# Autodesk Inventor assembly: Assembly_Cube_Z_Focus_MGN_NEMA_captive_v3
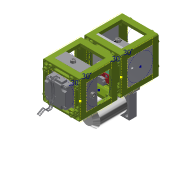
[picture p0: Inventor's stored thumbnail of the model, 180x180]
Saved by Autodesk Inventor 2022 (Build 260153000, 153)
## iProperties
Created: 2021-04-25
Part Number: Assembly_Cube_Z_Focus_MGN_NEMA_captive_v3
Document SubType Name: Assembly
Designer: diederichbenedict
Author: diederichbenedict
## Documents named in this file (17)
- C:\Users\diederichbenedict\Dropbox\Dokumente\Promotion\PROJECTS\UC2\02_CAD\INVENTOR\uc2_v3\Assembly_Cube_Z_Focus_MGN_NEMA_captive_v3.iam
- C:\Users\diederichbenedict\Dropbox\Dokumente\Promotion\PROJECTS\UC2\02_CAD\INVENTOR\uc2_v3\Assembly_Cube_empty_IM_v3.iam
- C:\Users\diederichbenedict\Dropbox\Dokumente\Promotion\PROJECTS\UC2\02_CAD\INVENTOR\uc2_v3\00_MGN12H, LINEAR GUIDE BLOCK.ipt
- C:\Users\diederichbenedict\Dropbox\Dokumente\Promotion\PROJECTS\UC2\02_CAD\INVENTOR\uc2_v3\00_NEMA11.ipt
- C:\Users\diederichbenedict\Dropbox\Dokumente\Promotion\PROJECTS\UC2\02_CAD\INVENTOR\uc2_v3\30_Cube_Z_Focus_MGN_NEMA_rail.ipt
- C:\Users\diederichbenedict\Dropbox\Dokumente\Promotion\PROJECTS\UC2\02_CAD\INVENTOR\uc2_v3\30_Cube_Z_Focus_MGN_NEMA_Motorsupport_centered.ipt
- C:\Users\diederichbenedict\Dropbox\Dokumente\Promotion\PROJECTS\UC2\02_CAD\INVENTOR\uc2_v3\30_Cube_Cube_Z_Focus_MGN_NEMA_belt_pushing_slide_v3.ipt
- C:\Users\diederichbenedict\Dropbox\Dokumente\Promotion\PROJECTS\UC2\02_CAD\INVENTOR\uc2_v3\30_Cube_Z_Focus_MGN_NEMA_base_belt_pushing_v3.ipt
- C:\Users\diederichbenedict\Dropbox\Dokumente\Promotion\PROJECTS\UC2\02_CAD\INVENTOR\uc2_v3\30_Cube_Z_Focus_MGN_NEMA_Motorcoupling_Captive_v3.ipt
- C:\Users\diederichbenedict\Documents\Inventor\Content Center Files\R2022\de-DE\DIN 912\DIN 912 - M3 x 0.5 x 30 x 18.ipt
- C:\Users\diederichbenedict\Documents\Inventor\Content Center Files\R2022\de-DE\DIN 912\DIN 912 - M3 x 0.5 x 16 x 14.75.ipt
- C:\Users\diederichbenedict\Documents\Inventor\Content Center Files\R2022\de-DE\DIN EN ISO 4032\DIN EN ISO 4032 - M3.ipt
- C:\Users\diederichbenedict\Documents\Inventor\Content Center Files\R2022\de-DE\DIN 912\DIN 912 - M3 x 0.5 x 8 x 6.75.ipt
- C:\Users\diederichbenedict\Dropbox\Dokumente\Promotion\PROJECTS\UC2\02_CAD\INVENTOR\uc2_v3\30_Cube_Z_Focus_MGN_NEMA_adapter_RMS.ipt
- C:\Users\diederichbenedict\Dropbox\Dokumente\Promotion\PROJECTS\UC2\02_CAD\INVENTOR\uc2_v3\00_Microscope_Objective_Lens10x.ipt
- C:\Users\diederichbenedict\Documents\Inventor\Content Center Files\R2022\de-DE\DIN 913\DIN 913 - M3 x 8.ipt
- C:\Users\diederichbenedict\Dropbox\Dokumente\Promotion\PROJECTS\UC2\02_CAD\INVENTOR\uc2_v3\30_Cube_Z_Focus_MGN_NEMA_Motorcoupling_captive_short_v3.ipt
## Components (29 placed, 16 different names)
1. 00_NEMA11:1 — Mate:9, Mate:10, Insert:3, Einfügen:25
2. 30_Cube_Z_Focus_MGN_NEMA_Motorsupport_centered:1 — Mate:6, Mate:7, Mate:8, Einfügen:6, Einfügen:7, Einfügen:8, Einfügen:9
3. 30_Cube_Z_Focus_MGN_NEMA_rail:1 — Insert:1, Angle:1, Mate:4, Einfügen:10
4. 00_MGN12H, LINEAR GUIDE BLOCK:1 — Angle:2, Mate:4, Mate:5, Insert:2, Angle:3
5. 30_Cube_Z_Focus_MGN_NEMA_base_belt_pushing_v3:1 — Mate:1, Mate:2, Mate:3, Insert:1, Mate:5, Mate:9, Einfügen:11, Einfügen:12, Einfügen:13
6. 30_Cube_Cube_Z_Focus_MGN_NEMA_belt_pushing_slide_v3:1 — Insert:2, Angle:3, Einfügen:14, Einfügen:15, Einfügen:17, Einfügen:18
7. 30_Cube_Z_Focus_MGN_NEMA_Motorcoupling_Captive_v3:1 — Insert:3, Passend:11, Einfügen:16, Einfügen:22, Einfügen:23, Einfügen:24
8. DIN 912 - ersetzt durch DIN EN ISO 4762 M3 x 30:1 — Passend:11
9. DIN 912 - ersetzt durch DIN EN ISO 4762 M3 x 16:1 — Einfügen:9
10. DIN 912 - ersetzt durch DIN EN ISO 4762 M3 x 16:2 — Einfügen:8
11. DIN 912 - ersetzt durch DIN EN ISO 4762 M3 x 16:3 — Einfügen:7
12. DIN 912 - ersetzt durch DIN EN ISO 4762 M3 x 16:4 — Einfügen:15
13. DIN 912 - ersetzt durch DIN EN ISO 4762 M3 x 16:5 — Einfügen:6
14. DIN EN ISO 4032 M3:1 — Einfügen:12
15. DIN EN ISO 4032 M3:3 — Einfügen:13
16. DIN EN ISO 4032 M3:4 — Einfügen:16
17. DIN 912 - ersetzt durch DIN EN ISO 4762 M3 x 8:1 — Einfügen:10
18. DIN 912 - ersetzt durch DIN EN ISO 4762 M3 x 8:2 — Einfügen:19
19. DIN 912 - ersetzt durch DIN EN ISO 4762 M3 x 8:3 — Einfügen:20
20. DIN 912 - ersetzt durch DIN EN ISO 4762 M3 x 8:4 — Einfügen:11
21. DIN 912 - ersetzt durch DIN EN ISO 4762 M3 x 16:6 — Einfügen:14
22. 30_Cube_Z_Focus_MGN_NEMA_adapter_RMS:1 — Einfügen:17, Einfügen:18, Einfügen:19, Einfügen:20, Einfügen:21
23. 00_Microscope_Objective_Lens10x:1 — Einfügen:21
24. DIN 913 M3 x 8:1 — Einfügen:24
25. DIN 913 M3 x 8:2 — Einfügen:23
26. DIN 913 M3 x 8:3 — Einfügen:22
27. 30_Cube_Z_Focus_MGN_NEMA_Motorcoupling_captive_short_v3:1 — Einfügen:25
28. Assembly_Cube_empty_IM_v3:4 [sub-assembly] — Mate:6, Mate:7, Mate:8, Mate:10
29. Assembly_Cube_empty_IM_v3:6 [sub-assembly] — Mate:1, Mate:2, Mate:3, Angle:1, Angle:2
## Component patterns: (2 elements, first: Assembly_Cube_empty_IM_v3:4)
## Relationships (37: Insert 23, Mate 11, Angle 3)
- Mate:1: 30_Cube_Z_Focus_MGN_NEMA_base_belt_pushing_v3:1 ↔ Assembly_Cube_empty_IM_v3:6
- Mate:2: 30_Cube_Z_Focus_MGN_NEMA_base_belt_pushing_v3:1 ↔ Assembly_Cube_empty_IM_v3:6
- Mate:3: 30_Cube_Z_Focus_MGN_NEMA_base_belt_pushing_v3:1 ↔ Assembly_Cube_empty_IM_v3:6
- Insert:1: 30_Cube_Z_Focus_MGN_NEMA_rail:1 ↔ 30_Cube_Z_Focus_MGN_NEMA_base_belt_pushing_v3:1
- Angle:1 (0 deg): 30_Cube_Z_Focus_MGN_NEMA_rail:1 ↔ Assembly_Cube_empty_IM_v3:6
- Angle:2 (0 deg): 00_MGN12H, LINEAR GUIDE BLOCK:1 ↔ Assembly_Cube_empty_IM_v3:6
- Mate:4: 30_Cube_Z_Focus_MGN_NEMA_rail:1 ↔ 00_MGN12H, LINEAR GUIDE BLOCK:1
- Mate:5: 00_MGN12H, LINEAR GUIDE BLOCK:1 ↔ 30_Cube_Z_Focus_MGN_NEMA_base_belt_pushing_v3:1
- Insert:2: 00_MGN12H, LINEAR GUIDE BLOCK:1 ↔ 30_Cube_Cube_Z_Focus_MGN_NEMA_belt_pushing_slide_v3:1
- Angle:3 (0 deg): 00_MGN12H, LINEAR GUIDE BLOCK:1 ↔ 30_Cube_Cube_Z_Focus_MGN_NEMA_belt_pushing_slide_v3:1
- Mate:6: 30_Cube_Z_Focus_MGN_NEMA_Motorsupport_centered:1 ↔ Assembly_Cube_empty_IM_v3:4
- Mate:7: 30_Cube_Z_Focus_MGN_NEMA_Motorsupport_centered:1 ↔ Assembly_Cube_empty_IM_v3:4
- Mate:8: 30_Cube_Z_Focus_MGN_NEMA_Motorsupport_centered:1 ↔ Assembly_Cube_empty_IM_v3:4
- Mate:9: 00_NEMA11:1 ↔ 30_Cube_Z_Focus_MGN_NEMA_base_belt_pushing_v3:1
- Mate:10: 00_NEMA11:1 ↔ Assembly_Cube_empty_IM_v3:4
- Insert:3: 00_NEMA11:1 ↔ 30_Cube_Z_Focus_MGN_NEMA_Motorcoupling_Captive_v3:1
- Einfügen:6 [Insert]: 30_Cube_Z_Focus_MGN_NEMA_Motorsupport_centered:1 ↔ DIN 912 - ersetzt durch DIN EN ISO 4762 M3 x 16:5
- Einfügen:7 [Insert]: 30_Cube_Z_Focus_MGN_NEMA_Motorsupport_centered:1 ↔ DIN 912 - ersetzt durch DIN EN ISO 4762 M3 x 16:3
- Einfügen:8 [Insert]: 30_Cube_Z_Focus_MGN_NEMA_Motorsupport_centered:1 ↔ DIN 912 - ersetzt durch DIN EN ISO 4762 M3 x 16:2
- Einfügen:9 [Insert]: 30_Cube_Z_Focus_MGN_NEMA_Motorsupport_centered:1 ↔ DIN 912 - ersetzt durch DIN EN ISO 4762 M3 x 16:1
- Einfügen:10 [Insert]: 30_Cube_Z_Focus_MGN_NEMA_rail:1 ↔ DIN 912 - ersetzt durch DIN EN ISO 4762 M3 x 8:1
- Einfügen:11 [Insert]: 30_Cube_Z_Focus_MGN_NEMA_base_belt_pushing_v3:1 ↔ DIN 912 - ersetzt durch DIN EN ISO 4762 M3 x 8:4
- Einfügen:12 [Insert]: 30_Cube_Z_Focus_MGN_NEMA_base_belt_pushing_v3:1 ↔ DIN EN ISO 4032 M3:1
- Einfügen:13 [Insert]: 30_Cube_Z_Focus_MGN_NEMA_base_belt_pushing_v3:1 ↔ DIN EN ISO 4032 M3:3
- Einfügen:14 [Insert]: 30_Cube_Cube_Z_Focus_MGN_NEMA_belt_pushing_slide_v3:1 ↔ DIN 912 - ersetzt durch DIN EN ISO 4762 M3 x 16:6
- Einfügen:15 [Insert]: 30_Cube_Cube_Z_Focus_MGN_NEMA_belt_pushing_slide_v3:1 ↔ DIN 912 - ersetzt durch DIN EN ISO 4762 M3 x 16:4
- Passend:11 [Mate]: 30_Cube_Z_Focus_MGN_NEMA_Motorcoupling_Captive_v3:1 ↔ DIN 912 - ersetzt durch DIN EN ISO 4762 M3 x 30:1
- Einfügen:16 [Insert]: 30_Cube_Z_Focus_MGN_NEMA_Motorcoupling_Captive_v3:1 ↔ DIN EN ISO 4032 M3:4
- Einfügen:17 [Insert]: 30_Cube_Cube_Z_Focus_MGN_NEMA_belt_pushing_slide_v3:1 ↔ 30_Cube_Z_Focus_MGN_NEMA_adapter_RMS:1
- Einfügen:18 [Insert]: 30_Cube_Cube_Z_Focus_MGN_NEMA_belt_pushing_slide_v3:1 ↔ 30_Cube_Z_Focus_MGN_NEMA_adapter_RMS:1
- Einfügen:19 [Insert]: DIN 912 - ersetzt durch DIN EN ISO 4762 M3 x 8:2 ↔ 30_Cube_Z_Focus_MGN_NEMA_adapter_RMS:1
- Einfügen:20 [Insert]: DIN 912 - ersetzt durch DIN EN ISO 4762 M3 x 8:3 ↔ 30_Cube_Z_Focus_MGN_NEMA_adapter_RMS:1
- Einfügen:21 [Insert]: 30_Cube_Z_Focus_MGN_NEMA_adapter_RMS:1 ↔ 00_Microscope_Objective_Lens10x:1
- Einfügen:22 [Insert]: 30_Cube_Z_Focus_MGN_NEMA_Motorcoupling_Captive_v3:1 ↔ DIN 913 M3 x 8:3
- Einfügen:23 [Insert]: 30_Cube_Z_Focus_MGN_NEMA_Motorcoupling_Captive_v3:1 ↔ DIN 913 M3 x 8:2
- Einfügen:24 [Insert]: 30_Cube_Z_Focus_MGN_NEMA_Motorcoupling_Captive_v3:1 ↔ DIN 913 M3 x 8:1
- Einfügen:25 [Insert]: 00_NEMA11:1 ↔ 30_Cube_Z_Focus_MGN_NEMA_Motorcoupling_captive_short_v3:1
